# Autodesk Inventor assembly: robot
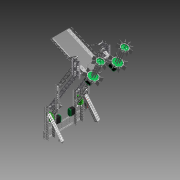
[picture p0: Inventor's stored thumbnail of the model, 180x180]
Saved by Autodesk Inventor 2014 SP1 (Build 180222100, 222)
## iProperties
Created: 2013-09-09
Part Number: robot
Document SubType Name: Assembly
Designer: Ryan
Author: Ryan
## Documents named in this file (14)
- C:\Users\Ryan\Desktop\pack and go\Workspaces\Workspace\toss up 1st A bot\manipulator\manipulator.iam
- C:\Users\Ryan\Desktop\pack and go\Workspaces\Workspace\toss up 1st A bot\toss up tower\tower1.iam
- C:\Users\Ryan\Desktop\pack and go\Workspaces\Workspace\toss up 1st A bot\toss up tower\encoder metal assembly.iam
- C:\Users\Ryan\Desktop\pack and go\Workspaces\Workspace\toss up 1st A bot\toss up tower\triangle support.iam
- C:\Users\Ryan\Desktop\pack and go\Workspaces\Workspace\toss up 1st A bot\toss up tower\back support.iam
- C:\Users\Ryan\Desktop\pack and go\Workspaces\Workspace\toss up 1st A bot\toss up tower\triangle support_MIR.iam
- C:\Users\Ryan\Desktop\pack and go\Workspaces\Workspace\toss up 1st A bot\6 bar\6 bar.iam
- C:\Users\Ryan\Desktop\pack and go\Workspaces\Workspace\toss up 1st A bot\6 bar\6 bar_MIR.iam
- C:\Users\Ryan\Desktop\pack and go\Workspaces\Workspace\toss up 1st A bot\toss up robot intake\intake.iam
- C:\Users\Ryan\Desktop\pack and go\Workspaces\Workspace\toss up 1st A bot\toss up robot intake\intake_MIR.iam
- C:\Users\Ryan\Desktop\pack and go\Workspaces\Workspace\toss up 1st A bot\toss up robot intake\flop down intake part.iam
- C:\Users\Ryan\Desktop\pack and go\Workspaces\Workspace\toss up 1st A bot\toss up robot intake\flop down intake part_MIR1.iam
- C:\Users\Ryan\Desktop\pack and go\Workspaces\Workspace\toss up 1st A bot\toss up robot intake\spinning part.iam
- C:\Users\Ryan\Desktop\pack and go\Workspaces\Workspace\toss up 1st A bot\toss up robot intake\polycarb.ipt
## Components (15 placed, 13 different names)
1. back support:1 [sub-assembly] — Mate:35, Flush:37, Flush:38, Mate:89, Flush:43, Flush:44
2. 6 bar:1 [sub-assembly] — Mate:69, Mate:70, Mate:71, Angle:3, Mate:93, Mate:94, Mate:95, Mate:96
3. 6 bar_MIR:1 [sub-assembly] — Mate:64, Mate:65, Mate:66, Mate:67, Mate:68, Mate:72, Mate:73, Mate:74, Angle:3
4. intake:1 [sub-assembly] — Mate:69, Mate:70, Mate:71, Mate:75, Mate:76, Mate:83, Mate:84
5. intake_MIR:1 [sub-assembly] — Mate:72, Mate:73, Mate:74, Mate:77, Mate:78, Flush:42, Mate:92
6. flop down intake part:1 [sub-assembly] — Mate:75, Mate:76, Angle:2, Mate:87, Mate:88
7. flop down intake part_MIR1:1 [sub-assembly] — Mate:77, Mate:78, Angle:1, Mate:85, Mate:86
8. spinning part:1 [sub-assembly] — Mate:85, Mate:86
9. spinning part:2 [sub-assembly] — Mate:87, Mate:88
10. polycarb:1 — Mate:83, Flush:42, Mate:84, Angle:1, Angle:2, Mate:92
11. tower1:2 [sub-assembly] — Mate:89, Flush:43, Flush:44, Mate:93, Mate:94, Mate:95, Mate:96
12. encoder metal assembly:1 [sub-assembly] — Mate:7, Mate:8, Mate:9
13. tower1:1 [sub-assembly] — Mate:7, Mate:8, Mate:9, Mate:21, Mate:35, Flush:37, Flush:38, Mate:49, Mate:50, Tangent:1, Mate:54, Mate:64, Mate:65, Mate:66, Mate:67, Mate:68
14. triangle support:1 [sub-assembly] — Mate:21, Mate:49, Mate:50, Tangent:1, Flush:40, Flush:41, Mate:54
15. triangle support_MIR:1 [sub-assembly] — Flush:40, Flush:41
## Relationships (46: Mate 35, Flush 7, Angle 3, Tangent 1)
- Mate:7: encoder metal assembly:1 ↔ tower1:1
- Mate:8: encoder metal assembly:1 ↔ tower1:1
- Mate:9 (2.3114 mm): encoder metal assembly:1 ↔ tower1:1
- Mate:21 (2.3114 mm): tower1:1 ↔ triangle support:1
- Mate:35: back support:1 ↔ tower1:1
- Flush:37: back support:1 ↔ tower1:1
- Flush:38: back support:1 ↔ tower1:1
- Mate:49 (2.3114 mm): tower1:1 ↔ triangle support:1
- Mate:50: tower1:1 ↔ triangle support:1
- Tangent:1 (90.0684 mm): tower1:1 ↔ triangle support:1
- Flush:40: triangle support:1 ↔ triangle support_MIR:1
- Flush:41: triangle support:1 ↔ triangle support_MIR:1
- Mate:54 (7.2898 mm): tower1:1 ↔ triangle support:1
- Mate:64: 6 bar_MIR:1 ↔ tower1:1
- Mate:65 (2.3114 mm): 6 bar_MIR:1 ↔ tower1:1
- Mate:66 (2.3114 mm): 6 bar_MIR:1 ↔ tower1:1
- Mate:67 (2.3114 mm): 6 bar_MIR:1 ↔ tower1:1
- Mate:68: 6 bar_MIR:1 ↔ tower1:1
- Mate:69: 6 bar:1 ↔ intake:1
- Mate:70: 6 bar:1 ↔ intake:1
- Mate:71: 6 bar:1 ↔ intake:1
- Mate:72: 6 bar_MIR:1 ↔ intake_MIR:1
- Mate:73: 6 bar_MIR:1 ↔ intake_MIR:1
- Mate:74: 6 bar_MIR:1 ↔ intake_MIR:1
- Mate:75: intake:1 ↔ flop down intake part:1
- Mate:76: intake:1 ↔ flop down intake part:1
- Mate:77: intake_MIR:1 ↔ flop down intake part_MIR1:1
- Mate:78: intake_MIR:1 ↔ flop down intake part_MIR1:1
- Mate:83: intake:1 ↔ polycarb:1
- Flush:42: intake_MIR:1 ↔ polycarb:1
- Mate:84: intake:1 ↔ polycarb:1
- Angle:1 (0 deg): flop down intake part_MIR1:1 ↔ polycarb:1
- Angle:2 (0 deg): flop down intake part:1 ↔ polycarb:1
- Mate:85: flop down intake part_MIR1:1 ↔ spinning part:1
- Mate:86: flop down intake part_MIR1:1 ↔ spinning part:1
- Mate:87: flop down intake part:1 ↔ spinning part:2
- Mate:88: flop down intake part:1 ↔ spinning part:2
- Mate:89: back support:1 ↔ tower1:2
- Flush:43: back support:1 ↔ tower1:2
- Flush:44: back support:1 ↔ tower1:2
- Mate:92: intake_MIR:1 ↔ polycarb:1
- Angle:3 (0 deg): 6 bar:1 ↔ 6 bar_MIR:1
- Mate:93: 6 bar:1 ↔ tower1:2
- Mate:94: 6 bar:1 ↔ tower1:2
- Mate:95 (2.3114 mm): 6 bar:1 ↔ tower1:2
- Mate:96 (2.3114 mm): 6 bar:1 ↔ tower1:2
## Named parameters: q = 2.3114 mm
